# Autodesk Inventor assembly: Сборка2
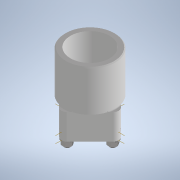
[picture p0: Inventor's stored thumbnail of the model, 180x180]
Saved by Autodesk Inventor 2021 (Build 250183000, 183)
## iProperties
Created: 2020-05-07
Part Number: Сборка2
Document SubType Name: Assembly
Designer: 2000
Mass: 959.878 g
Surface Area: 1498.52 cm^2
Volume: 720.008 cm^3
Density: 1.33315 g/cm^3
Author: 2000
## Documents named in this file (6)
- C:\Users\2000\Desktop\Сборка2.iam
- C:\Users\2000\Desktop\Пункт 1(чё там считать).ipt
- C:\Users\2000\Desktop\Деталь2.ipt
- C:\Users\2000\Documents\Inventor\Content Center Files\R2021\ru-RU\GOST 11371-78  A\Шайба 12 ГОСТ 11371-78.ipt
- C:\Users\2000\Documents\Inventor\Content Center Files\R2021\ru-RU\Nut GOST ISO 4032-2014\M12-6H ГОСТ ISO 4032-2014.ipt
- C:\Users\2000\Documents\Inventor\Content Center Files\R2021\ru-RU\Stud GOST 22036-76\Шпилька M12-6g×32 ГОСТ 22036-76.ipt
## Components (14 placed, 5 different names)
1. Пункт 1(чё там считать):1 — Жесткий:1, Вставка:1, Вставка:3, Вставка:4, Вставка:5
2. Деталь2:1 — Жесткий:1, Совмещение:2, Совмещение:4, Вставка:6, Вставка:7
3. Шпилька ГОСТ 22036-76 M12-6g×32:1 — Вставка:1, Совмещение:1
4. Шпилька ГОСТ 22036-76 M12-6g×32:3 — Вставка:4, Совмещение:3
5. Шпилька ГОСТ 22036-76 M12-6g×32:4 — Вставка:5
6. Шпилька ГОСТ 22036-76 M12-6g×32:2 — Вставка:3
7. Шайба  ГОСТ 11371-78 13:1 — Совмещение:1, Совмещение:2, Вставка:2
8. Гайка ГОСТ ISO 4032-2014 M12:1 — Вставка:2
9. Шайба  ГОСТ 11371-78 13:2 — Совмещение:3, Совмещение:4, Вставка:10
10. Шайба  ГОСТ 11371-78 13:3 — Вставка:6, Вставка:8
11. Шайба  ГОСТ 11371-78 13:4 — Вставка:7, Вставка:9
12. Гайка ГОСТ ISO 4032-2014 M12:2 — Вставка:8
13. Гайка ГОСТ ISO 4032-2014 M12:3 — Вставка:9
14. Гайка ГОСТ ISO 4032-2014 M12:4 — Вставка:10
## Relationships (15: Insert 10, Mate 4, WeldJoint 1)
- Жесткий:1 [WeldJoint]: Пункт 1(чё там считать):1 ↔ Деталь2:1
- Вставка:1 [Insert] (10.5 mm): Пункт 1(чё там считать):1 ↔ Шпилька ГОСТ 22036-76 M12-6g×32:1
- Совмещение:1 [Mate]: Шпилька ГОСТ 22036-76 M12-6g×32:1 ↔ Шайба  ГОСТ 11371-78 13:1
- Совмещение:2 [Mate]: Деталь2:1 ↔ Шайба  ГОСТ 11371-78 13:1
- Вставка:2 [Insert]: Шайба  ГОСТ 11371-78 13:1 ↔ Гайка ГОСТ ISO 4032-2014 M12:1
- Вставка:3 [Insert] (10.5 mm): Пункт 1(чё там считать):1 ↔ Шпилька ГОСТ 22036-76 M12-6g×32:2
- Вставка:4 [Insert] (10.5 mm): Пункт 1(чё там считать):1 ↔ Шпилька ГОСТ 22036-76 M12-6g×32:3
- Вставка:5 [Insert] (10.5 mm): Пункт 1(чё там считать):1 ↔ Шпилька ГОСТ 22036-76 M12-6g×32:4
- Совмещение:3 [Mate]: Шпилька ГОСТ 22036-76 M12-6g×32:3 ↔ Шайба  ГОСТ 11371-78 13:2
- Совмещение:4 [Mate]: Деталь2:1 ↔ Шайба  ГОСТ 11371-78 13:2
- Вставка:6 [Insert]: Деталь2:1 ↔ Шайба  ГОСТ 11371-78 13:3
- Вставка:7 [Insert]: Деталь2:1 ↔ Шайба  ГОСТ 11371-78 13:4
- Вставка:8 [Insert]: Шайба  ГОСТ 11371-78 13:3 ↔ Гайка ГОСТ ISO 4032-2014 M12:2
- Вставка:9 [Insert]: Шайба  ГОСТ 11371-78 13:4 ↔ Гайка ГОСТ ISO 4032-2014 M12:3
- Вставка:10 [Insert]: Шайба  ГОСТ 11371-78 13:2 ↔ Гайка ГОСТ ISO 4032-2014 M12:4
